# Autodesk Inventor assembly: SA-117_v0.2
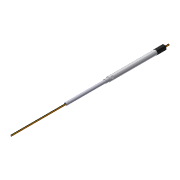
[picture p0: Inventor's stored thumbnail of the model, 180x180]
Saved by Autodesk Inventor 2019.3 (Build 233278000, 278)
## iProperties
Created: 2018-11-30
Part Number: SA-117_v0.2
Document SubType Name: Assembly
Designer: ddeboer
Author: ddeboer
## Documents named in this file (5)
- C:\Users\Kathryn Rosie\Google Drive\HERA\Feed\CAD\SA-117_v0.2.iam
- C:\Users\Kathryn Rosie\Google Drive\HERA\Feed\CAD\Dave Conduit 20190117\sch40_conduit-master\outer_assy.iam
- C:\Users\Kathryn Rosie\Google Drive\HERA\Feed\CAD\Dave Conduit 20190117\sch40_conduit-master\inner_assy.iam
- C:\Users\Kathryn Rosie\Google Drive\HERA\Feed\CAD\Dave Conduit 20190117\sch40_conduit-master\insert.ipt
- C:\Users\Kathryn Rosie\Google Drive\HERA\Feed\CAD\Dave Conduit 20190117\sch40_conduit-master\cables.ipt
## Components (4 placed, 4 different names)
1. outer_assy:1 [sub-assembly] — Insert:4
2. inner_assy:1 [sub-assembly] — Insert:2, Mate:1, Insert:3, Insert:4
3. insert:1 — Insert:2, Mate:1
4. cables:1 — Insert:3
## Relationships (4: Insert 3, Mate 1)
- Insert:2: inner_assy:1 ↔ insert:1
- Mate:1: inner_assy:1 ↔ insert:1
- Insert:3 (-60 mm): inner_assy:1 ↔ cables:1
- Insert:4 (-10 mm): outer_assy:1 ↔ inner_assy:1
